# Autodesk Inventor assembly: Z_GANTRY
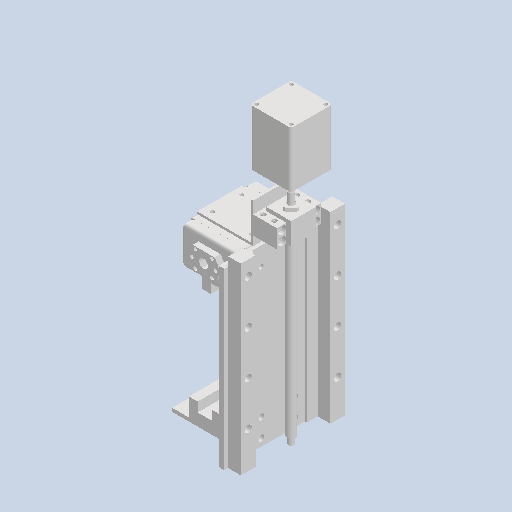
[picture p0: Inventor's stored thumbnail of the model, 512x512]
Saved by Autodesk Inventor 2023 (Build 270158000, 158)
## iProperties
Created: 2022-05-07
Part Number: Z_GANTRY
Document SubType Name: Assembly
Designer: plebbb
Author: plebbb
## Documents named in this file (11)
- D:\Users\plebbb\Desktop\CNC_Project\Z_GANTRY.iam
- D:\Users\plebbb\Desktop\CNC_Project\Ballscrew_Assembly_1204.iam
- D:\Users\plebbb\Desktop\CNC_Project\Flat_Plate.ipt
- D:\Users\plebbb\Desktop\CNC_Project\HGW20CC_Rail_300mm.ipt
- D:\Users\plebbb\Desktop\CNC_Project\Rail_Spacer_Plate.ipt
- D:\Users\plebbb\Desktop\CNC_Project\SFU1204-300.ipt
- D:\Users\plebbb\Desktop\CNC_Project\Nema23.ipt
- D:\Users\plebbb\Desktop\CNC_Project\BK10.ipt
- D:\Users\plebbb\Desktop\CNC_Project\Z_Screw_Holder_Bracket.ipt
- D:\Users\plebbb\Desktop\CNC_Project\L_Bracketr.ipt
- D:\Users\plebbb\Desktop\CNC_Project\HGW20CC_Slider.ipt
## Components (12 placed, 10 different names)
1. Ballscrew_Assembly_1204:1 [sub-assembly]
2. Flat_Plate:1
3. HGW20CC_Rail_300mm:1
4. HGW20CC_Rail_300mm:2
5. Rail_Spacer_Plate:1
6. SFU1204-300:1
7. Nema23:1
8. BK10:1
9. Z_Screw_Holder_Bracket:1
10. Rail_Spacer_Plate:2
11. L_Bracketr:1
12. HGW20CC_Slider:1
## Relationships (32: Mate 21, Flush 9, Angle 2)
- [Mate]: Ballscrew_Assembly_1204:1 ↔ Flat_Plate:1
- [Flush]: Ballscrew_Assembly_1204:1 ↔ Flat_Plate:1
- [Mate]: HGW20CC_Rail_300mm:1 ↔ Rail_Spacer_Plate:1
- [Angle] (0 deg): HGW20CC_Rail_300mm:1 ↔ HGW20CC_Rail_300mm:2
- [Angle] (0 deg): Flat_Plate:1 ↔ HGW20CC_Rail_300mm:1
- [Flush]: HGW20CC_Rail_300mm:1 ↔ HGW20CC_Rail_300mm:2
- [Flush]: Flat_Plate:1 ↔ Rail_Spacer_Plate:1
- [Mate]: Flat_Plate:1 ↔ Rail_Spacer_Plate:1
- [Flush]: Flat_Plate:1 ↔ Rail_Spacer_Plate:1
- [Flush]: Flat_Plate:1 ↔ HGW20CC_Rail_300mm:1
- [Flush] (-5.2 mm): Flat_Plate:1 ↔ HGW20CC_Rail_300mm:1
- [Mate]: Ballscrew_Assembly_1204:1 ↔ Flat_Plate:1
- [Mate]: Ballscrew_Assembly_1204:1 ↔ Flat_Plate:1
- [Flush]: Flat_Plate:1 ↔ SFU1204-300:1
- [Mate]: SFU1204-300:1 ↔ BK10:1
- [Mate]: SFU1204-300:1 ↔ BK10:1
- [Mate]: Ballscrew_Assembly_1204:1 ↔ Z_Screw_Holder_Bracket:1
- [Mate]: Ballscrew_Assembly_1204:1 ↔ Z_Screw_Holder_Bracket:1
- [Mate]: Ballscrew_Assembly_1204:1 ↔ Z_Screw_Holder_Bracket:1
- [Mate]: BK10:1 ↔ Z_Screw_Holder_Bracket:1
- [Mate]: SFU1204-300:1 ↔ Nema23:1
- [Mate]: SFU1204-300:1 ↔ Nema23:1
- [Mate]: HGW20CC_Rail_300mm:2 ↔ Rail_Spacer_Plate:2
- [Mate]: Flat_Plate:1 ↔ Rail_Spacer_Plate:2
- [Flush]: Flat_Plate:1 ↔ Rail_Spacer_Plate:2
- [Flush]: Flat_Plate:1 ↔ Rail_Spacer_Plate:2
- [Mate]: Flat_Plate:1 ↔ L_Bracketr:1
- [Mate]: Flat_Plate:1 ↔ L_Bracketr:1
- [Mate]: Flat_Plate:1 ↔ L_Bracketr:1
- [Mate]: L_Bracketr:1 ↔ HGW20CC_Slider:1
- [Mate]: L_Bracketr:1 ↔ HGW20CC_Slider:1
- [Mate]: L_Bracketr:1 ↔ HGW20CC_Slider:1
